# Autodesk Inventor assembly: mini pulley assembly
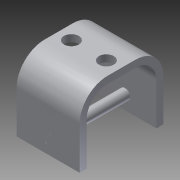
[picture p0: Inventor's stored thumbnail of the model, 180x180]
Saved by Autodesk Inventor 2013 (Build 170138000, 138)
## iProperties
Created: 2013-01-27
Part Number: mini pulley assembly
Document SubType Name: Assembly
Designer: Arpan
Author: Arpan
## Documents named in this file (3)
- C:\Users\Arpan\Documents\GitHub\frc2013CAD\Cimber actual\mini pulley assembly.iam
- C:\Users\Arpan\Documents\GitHub\frc2013CAD\Cimber actual\pulley mount.ipt
- C:\Users\Arpan\Documents\GitHub\frc2013CAD\Cimber actual\1.5 inch shaft.ipt
## Components (2 placed, 2 different names)
1. pulley mount:1 — Mate:1, Flush:1
2. 1.5 inch shaft:1 — Mate:1, Flush:1
## Relationships (2: Mate 1, Flush 1)
- Mate:1: pulley mount:1 ↔ 1.5 inch shaft:1
- Flush:1: pulley mount:1 ↔ 1.5 inch shaft:1
